# Autodesk Inventor assembly: SingleSpeedDriveTrain
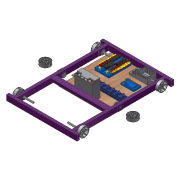
[picture p0: Inventor's stored thumbnail of the model, 180x180]
Saved by Autodesk Inventor 2012 (Build 160160000, 160)
## iProperties
Created: 2012-11-20
Part Number: SingleSpeedDriveTrain
Document SubType Name: Assembly
Designer: JesseK
Author: JesseK
## Documents named in this file (7)
- Z:\UserData\Documents\Inventor\team1885frc\Robot2013\DriveTrainProto\SingleSpeedDriveTrain.iam
- Z:\UserData\Documents\Inventor\team1885frc\Robot2013\DriveTrainProto\DriveTrainFrame.iam
- Z:\UserData\Documents\Inventor\team1885frc\Robot2013\DriveTrainProto\OuterAxle.ipt
- Z:\UserData\Documents\Inventor\team1885frc\AndyMark\Sprocket_Num25_22T_0.5bore.ipt
- Z:\UserData\Documents\Inventor\team1885frc\Robot2013\DriveTrainProto\ElectronicsBoard.iam
- Z:\UserData\Documents\Inventor\team1885frc\Electronics\Battery.ipt
- Z:\UserData\Documents\Inventor\team1885frc\AndyMark\4 Perf ThruTread 500 Hex.ipt
## Components (17 placed, 6 different names)
1. DriveTrainFrame:1 [sub-assembly] — Mate:35, Mate:37, Mate:39, Mate:41, Mate:60, Mate:61, Mate:62, Mate:64, Mate:65, Mate:66, Mate:69, Mate:70, Mate:71, Mate:72, Mate:75, Mate:76, Mate:77, Mate:80, Mate:81, Mate:82
2. Sprocket_Num25_22T_0.5bore:1 — Mate:35
3. Sprocket_Num25_22T_0.5bore:2 — Mate:37
4. Sprocket_Num25_22T_0.5bore:3 — Mate:39
5. Sprocket_Num25_22T_0.5bore:4 — Mate:41
6. ElectronicsBoard:1 [sub-assembly] — Mate:60, Mate:61, Mate:62, Mate:63
7. Battery:1 — Mate:63, Mate:64
8. 4 Perf ThruTread 500 Hex:1 — Flush:1, Mate:67, Mate:68, Mate:69
9. 4 Perf ThruTread 500 Hex:2
10. 4 Perf ThruTread 500 Hex:3 — Mate:82, Flush:4, Mate:83, Mate:84
11. 4 Perf ThruTread 500 Hex:4 — Mate:77, Flush:3, Mate:78, Mate:79
12. 4 Perf ThruTread 500 Hex:5
13. 4 Perf ThruTread 500 Hex:6 — Mate:72, Flush:2, Mate:73, Mate:74
14. OuterAxle:1 — Mate:65, Mate:66, Flush:1, Mate:67, Mate:68
15. OuterAxle:2 — Mate:80, Mate:81, Flush:4, Mate:83, Mate:84
16. OuterAxle:3 — Mate:75, Mate:76, Flush:3, Mate:78, Mate:79
17. OuterAxle:4 — Mate:70, Mate:71, Flush:2, Mate:73, Mate:74
## Relationships (33: Mate 29, Flush 4)
- Mate:35: DriveTrainFrame:1 ↔ Sprocket_Num25_22T_0.5bore:1
- Mate:37 (3.175 mm): DriveTrainFrame:1 ↔ Sprocket_Num25_22T_0.5bore:2
- Mate:39: DriveTrainFrame:1 ↔ Sprocket_Num25_22T_0.5bore:3
- Mate:41 (3.175 mm): DriveTrainFrame:1 ↔ Sprocket_Num25_22T_0.5bore:4
- Mate:60: DriveTrainFrame:1 ↔ ElectronicsBoard:1
- Mate:61: DriveTrainFrame:1 ↔ ElectronicsBoard:1
- Mate:62: DriveTrainFrame:1 ↔ ElectronicsBoard:1
- Mate:63: ElectronicsBoard:1 ↔ Battery:1
- Mate:64: DriveTrainFrame:1 ↔ Battery:1
- Mate:65: DriveTrainFrame:1 ↔ OuterAxle:1
- Mate:66: DriveTrainFrame:1 ↔ OuterAxle:1
- Flush:1: 4 Perf ThruTread 500 Hex:1 ↔ OuterAxle:1
- Mate:67: 4 Perf ThruTread 500 Hex:1 ↔ OuterAxle:1
- Mate:68: 4 Perf ThruTread 500 Hex:1 ↔ OuterAxle:1
- Mate:69 (3.175 mm): DriveTrainFrame:1 ↔ 4 Perf ThruTread 500 Hex:1
- Mate:70: DriveTrainFrame:1 ↔ OuterAxle:4
- Mate:71: DriveTrainFrame:1 ↔ OuterAxle:4
- Mate:72 (3.175 mm): DriveTrainFrame:1 ↔ 4 Perf ThruTread 500 Hex:6
- Flush:2: 4 Perf ThruTread 500 Hex:6 ↔ OuterAxle:4
- Mate:73: 4 Perf ThruTread 500 Hex:6 ↔ OuterAxle:4
- Mate:74: 4 Perf ThruTread 500 Hex:6 ↔ OuterAxle:4
- Mate:75: DriveTrainFrame:1 ↔ OuterAxle:3
- Mate:76: DriveTrainFrame:1 ↔ OuterAxle:3
- Mate:77 (3.175 mm): DriveTrainFrame:1 ↔ 4 Perf ThruTread 500 Hex:4
- Flush:3: 4 Perf ThruTread 500 Hex:4 ↔ OuterAxle:3
- Mate:78: 4 Perf ThruTread 500 Hex:4 ↔ OuterAxle:3
- Mate:79: 4 Perf ThruTread 500 Hex:4 ↔ OuterAxle:3
- Mate:80: DriveTrainFrame:1 ↔ OuterAxle:2
- Mate:81: DriveTrainFrame:1 ↔ OuterAxle:2
- Mate:82 (3.175 mm): DriveTrainFrame:1 ↔ 4 Perf ThruTread 500 Hex:3
- Flush:4: 4 Perf ThruTread 500 Hex:3 ↔ OuterAxle:2
- Mate:83: 4 Perf ThruTread 500 Hex:3 ↔ OuterAxle:2
- Mate:84: 4 Perf ThruTread 500 Hex:3 ↔ OuterAxle:2
